# Autodesk Inventor assembly: GoPro
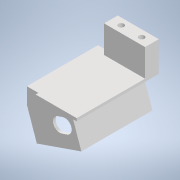
[picture p0: Inventor's stored thumbnail of the model, 180x180]
Saved by Autodesk Inventor 2020 (Build 240168000, 168)
## iProperties
Created: 2020-02-19
Part Number: GoPro
Document SubType Name: Assembly
Designer: maple
Author: maple
## Documents named in this file (3)
- C:\Users\maple\Documents\GitHub\3D-Models\Personal Project\GoPro\GoPro.iam
- C:\Users\maple\Documents\GitHub\3D-Models\Personal Project\GoPro\Base.ipt
- C:\Users\maple\Documents\GitHub\3D-Models\Personal Project\GoPro\GoProCase.ipt
## Components (2 placed, 2 different names)
1. GoProCase:1 — Flush:1, Mate:1, Mate:2
2. Base:1 — Flush:1, Mate:1, Mate:2
## Relationships (3: Mate 2, Flush 1)
- Flush:1: GoProCase:1 ↔ Base:1
- Mate:1: GoProCase:1 ↔ Base:1
- Mate:2: GoProCase:1 ↔ Base:1
